# Autodesk Inventor assembly: black-suspension
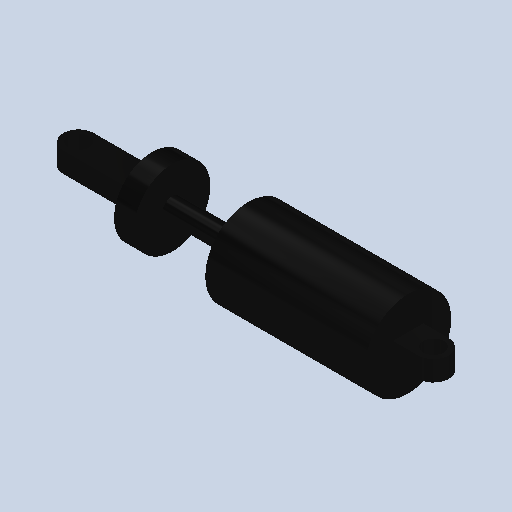
[picture p0: Inventor's stored thumbnail of the model, 512x512]
Saved by Autodesk Inventor 2025.1 (Build 291241000, 241)
## iProperties
Created: 2023-11-21
Part Number: black-suspension
Document SubType Name: Assembly
Designer: haruy
Author: haruy
## Documents named in this file (3)
- C:\Users\haruy\Documents\ロボコン\NHK2025\cad\000_parts\サスペンション\black-suspension.iam
- C:\Users\haruy\Documents\ロボコン\NHK2025\cad\000_parts\サスペンション\black-suspension-top.ipt
- C:\Users\haruy\Documents\ロボコン\NHK2025\cad\000_parts\サスペンション\black-suspension-under.ipt
## Components (2 placed, 2 different names)
1. black-suspension-top:1 — 円柱状:1, 角度:1
2. black-suspension-under:1 — 円柱状:1, 角度:1
## Relationships (2: CylindricalJoint 1, Angle 1)
- 円柱状:1 [CylindricalJoint]: black-suspension-top:1 ↔ black-suspension-under:1
- 角度:1 [Angle] (0 deg): black-suspension-top:1 ↔ black-suspension-under:1
